# Autodesk Inventor assembly: Batteriepack
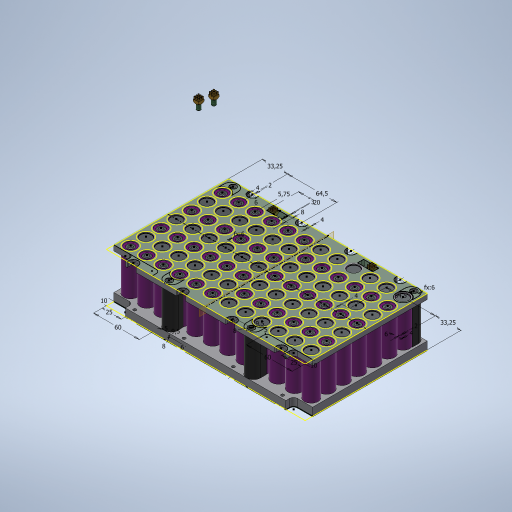
[picture p0: Inventor's stored thumbnail of the model, 512x512]
Saved by Autodesk Inventor 2024 (Build 280153000, 153)
## iProperties
Created: 2025-03-26
Part Number: Batteriepack
Document SubType Name: Assembly
Designer: David Lill
Author: David Lill
## Documents named in this file (8)
- C:\Users\Angela Ogrenda\Documents\Batterie_Konstruktion\E-16 Batterie\Batteriepack.iam
- C:\Users\Angela Ogrenda\Documents\Backup Inventor\Platte1.ipt
- C:\Users\Angela Ogrenda\Documents\Backup Inventor\18650.ipt
- C:\Users\Angela Ogrenda\Documents\Backup Inventor\REDCUBEM7x7.ipt
- C:\Users\Angela Ogrenda\Documents\Backup Inventor\Abstandhalter.ipt
- C:\Users\Angela Ogrenda\Documents\Backup Inventor\Platte2.ipt
- C:\Users\Angela Ogrenda\Documents\Backup Inventor\PCB.ipt
- C:\Users\Angela Ogrenda\Documents\Backup Inventor\REDCUBEM7x7_MIR.ipt
## Components (96 placed, 7 different names)
1. Platte1:3 — Einfügen:5, Einfügen:6, Einfügen:7, Einfügen:8, Fluchtend:1, Einfügen:10, Einfügen:11, Passend:5, Passend:6, Passend:7, Passend:8, Fluchtend:2, Passend:9
2. REDCUBEM7x7:1 — Passend:7, Passend:8, Fluchtend:2
3. Abstandhalter:1
4. Abstandhalter:2
5. Platte2:2 — Fluchtend:1, Einfügen:9, Passend:3, Passend:4
6. Abstandhalter:3 — Einfügen:9, Einfügen:10, Passend:1
7. Abstandhalter:6 — Einfügen:11, Passend:2
8. REDCUBEM7x7:3
9. REDCUBEM7x7:4
10. PCB:1 — Passend:5, Passend:6, Winkel:1
11. PCB:2 — Passend:3, Passend:4
12. REDCUBEM7x7_MIR:1
13. 18650:1 — Einfügen:5
14. 18650:4 — Einfügen:8
15. 18650:5
16. 18650:6
17. 18650:7
18. 18650:8
19. 18650:9
20. 18650:10
21. 18650:11
22. 18650:12
23. 18650:13
24. 18650:14
25. 18650:25
26. 18650:26
27. 18650:27
28. 18650:28
29. 18650:29
30. 18650:30
31. 18650:31
32. 18650:32
33. 18650:33
34. 18650:34
35. 18650:35
36. 18650:36
37. 18650:37
38. 18650:38
39. 18650:39
40. 18650:40
41. 18650:41
42. 18650:42
43. 18650:43
44. 18650:44
45. 18650:45
46. 18650:46
47. 18650:47
48. 18650:48
49. 18650:49 — Passend:2
50. 18650:50
51. 18650:51
52. 18650:52
53. 18650:53
54. 18650:54
55. 18650:55
56. 18650:56
57. 18650:57
58. 18650:58
59. 18650:59
60. 18650:60 — Passend:1
61. 18650:2 — Einfügen:7
62. 18650:3 — Einfügen:6
63. 18650:15
64. 18650:16
65. 18650:17
66. 18650:18
67. 18650:19
68. 18650:20
69. 18650:21
70. 18650:22
71. 18650:23
72. 18650:24
73. 18650:61
74. 18650:62
75. 18650:63
76. 18650:64
77. 18650:65
78. 18650:66
79. 18650:67
80. 18650:68
81. 18650:69
82. 18650:70
83. 18650:71
84. 18650:72
85. 18650:73
86. 18650:74
87. 18650:75
88. 18650:76
89. 18650:77
90. 18650:78
91. 18650:79
92. 18650:80
93. 18650:81
94. 18650:82
95. 18650:83
96. 18650:84
## Component patterns: (4 elements), (3 elements), (6 elements, first: 18650:1 + 18650:4), Komponentenanordnung 5:2 (6 elements), Komponentenanordnung 5:3 (6 elements), Komponentenanordnung 5:4 (6 elements), (6 elements, first: 18650:2 + 18650:3), Komponentenanordnung 6:2 (6 elements), Komponentenanordnung 6:3 (6 elements)
## Relationships (19: Mate 9, Insert 7, Flush 2, Angle 1)
- Einfügen:5 [Insert]: Platte1:3 ↔ 18650:1
- Einfügen:6 [Insert]: Platte1:3 ↔ 18650:3
- Einfügen:7 [Insert]: Platte1:3 ↔ 18650:2
- Einfügen:8 [Insert]: Platte1:3 ↔ 18650:4
- Fluchtend:1 [Flush]: Platte1:3 ↔ Platte2:2
- Einfügen:9 [Insert]: Platte2:2 ↔ Abstandhalter:3
- Einfügen:10 [Insert]: Platte1:3 ↔ Abstandhalter:3
- Passend:1 [Mate]: Abstandhalter:3 ↔ 18650:60
- Einfügen:11 [Insert]: Platte1:3 ↔ Abstandhalter:6
- Passend:2 [Mate]: Abstandhalter:6 ↔ 18650:49
- Passend:3 [Mate]: Platte2:2 ↔ PCB:2
- Passend:4 [Mate]: Platte2:2 ↔ PCB:2
- Passend:5 [Mate]: Platte1:3 ↔ PCB:1
- Passend:6 [Mate]: Platte1:3 ↔ PCB:1
- Passend:7 [Mate]: Platte1:3 ↔ REDCUBEM7x7:1
- Passend:8 [Mate] (10.75 mm): Platte1:3 ↔ REDCUBEM7x7:1
- Fluchtend:2 [Flush] (7 mm): Platte1:3 ↔ REDCUBEM7x7:1
- Passend:9 [Mate]: Platte1:3
- Winkel:1 [Angle] (0 deg): PCB:1
